# Autodesk Inventor assembly: nozzle-assembly
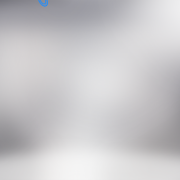
[picture p0: Inventor's stored thumbnail of the model, 180x180]
Saved by Autodesk Inventor 2016 (Build 200138000, 138)
## iProperties
Created: 2015-05-09
Part Number: nozzle-assembly
Document SubType Name: Assembly
Designer: ax
Mass: 27.77 g
Surface Area: 31.6175 cm^2
Volume: 3.41623 cm^3
Density: 8.12884 g/cm^3
Author: ax
## Documents named in this file (3)
- C:\Users\as\Documents\Inventor\mintplacer-export\nozzle-assembly.iam
- C:\Users\as\Documents\Inventor\mintplacer-export\nozzle-base.ipt
- C:\Users\as\Documents\Inventor\mintplacer-export\nozzle-tip1-0402.ipt
## Components (2 placed, 2 different names)
1. nozzle-base:1 — Flush:1
2. nozzle-tip1-0402:1 — Flush:1
## Relationships (1: Flush 1)
- Flush:1: nozzle-base:1 ↔ nozzle-tip1-0402:1
